# Autodesk Inventor assembly: SolarPanel
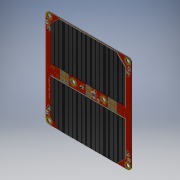
[picture p0: Inventor's stored thumbnail of the model, 180x180]
Saved by Autodesk Inventor 2018 (Build 220112000, 112)
## iProperties
Created: 2018-11-29
Part Number: SolarPanel
Document SubType Name: Assembly
Designer: Bradley
Author: Bradley
## Documents named in this file (32)
- C:\Users\Bradley\Documents\GitHub\CougSat1-Hardware\CougSat1-PowerBoard\CADModel\Native\SolarPanel.iam
- C:\Users\Bradley\Documents\GitHub\CougSat1-Hardware\CougSat1-PowerBoard\CADModel\Native\SolarPanel_PCB.ipt
- C:\Users\Bradley\Documents\GitHub\Resources\SupplierDocuments\04 - Connectors SMT\04-0001\04-0001.iam
- C:\Users\Bradley\Documents\GitHub\Resources\SupplierDocuments\04 - Connectors SMT\04-0007\04-0007.iam
- C:\Users\Bradley\Documents\GitHub\Resources\SupplierDocuments\26 - Resistor Misc\26-0008\26-0008.ipt
- C:\Users\Bradley\Documents\GitHub\Resources\SupplierDocuments\02 - Solar Cell\02-0001\02-0001.ipt
- C:\Users\Bradley\Documents\GitHub\Resources\SupplierDocuments\34 - Inductor 3225 and larger\34-103A\34-103A.ipt
- C:\Users\Bradley\Documents\GitHub\Resources\SupplierDocuments\66 - Sensor\66-0003\66-0003.ipt
- C:\Users\Bradley\Documents\GitHub\Resources\SupplierDocuments\21 - Resistor 1608\21-0000\21-0000.ipt
- C:\Users\Bradley\Documents\GitHub\Resources\SupplierDocuments\21 - Resistor 1608\21-1201\21-1201.ipt
- C:\Users\Bradley\Documents\GitHub\Resources\SupplierDocuments\21 - Resistor 1608\21-1001\21-1001.ipt
- C:\Users\Bradley\Documents\GitHub\Resources\SupplierDocuments\36 - Ferrite\36-152A\36-152A.ipt
- C:\Users\Bradley\Documents\GitHub\Resources\SupplierDocuments\11 - Capacitor Ceramic 1608\11-102A\11-102A.ipt
- C:\Users\Bradley\Documents\GitHub\Resources\SupplierDocuments\21 - Resistor 1608\21-2201\21-2201.ipt
- C:\Users\Bradley\Documents\GitHub\Resources\SupplierDocuments\16 - Capacitor Tantalum SMT\16-475A\16-475A.ipt
- C:\Users\Bradley\Documents\GitHub\Resources\SupplierDocuments\13 - Capacitor Ceramic 3216\13-475A\13-475A.ipt
- C:\Users\Bradley\Documents\GitHub\Resources\SupplierDocuments\23 - Resistor 3216\23-5m00\23-5m00.ipt
- C:\Users\Bradley\Documents\GitHub\Resources\SupplierDocuments\11 - Capacitor Ceramic 1608\11-106A\11-106A.ipt
- C:\Users\Bradley\Documents\GitHub\Resources\SupplierDocuments\13 - Capacitor Ceramic 3216\13-106A\13-106A.ipt
- C:\Users\Bradley\Documents\GitHub\Resources\SupplierDocuments\21 - Resistor 1608\21-1002\21-1002.ipt
- C:\Users\Bradley\Documents\GitHub\Resources\SupplierDocuments\23 - Resistor 3216\23-12m0\23-12m0.ipt
- C:\Users\Bradley\Documents\GitHub\Resources\SupplierDocuments\16 - Capacitor Tantalum SMT\16-476A\16-476A.ipt
- C:\Users\Bradley\Documents\GitHub\Resources\SupplierDocuments\26 - Resistor Misc\26-0005\26-0005.ipt
- C:\Users\Bradley\Documents\GitHub\Resources\SupplierDocuments\11 - Capacitor Ceramic 1608\11-104A\11-104A.ipt
- C:\Users\Bradley\Documents\GitHub\Resources\SupplierDocuments\21 - Resistor 1608\21-3603\21-3603.ipt
- C:\Users\Bradley\Documents\GitHub\Resources\SupplierDocuments\21 - Resistor 1608\21-8203\21-8203.ipt
- C:\Users\Bradley\Documents\GitHub\Resources\SupplierDocuments\27 - Conversion IC\27-0003\27-0003.ipt
- C:\Users\Bradley\Documents\GitHub\Resources\SupplierDocuments\08 - Amplifier (excluding RF)\08-0002\08-0002.ipt
- C:\Users\Bradley\Documents\GitHub\Resources\SupplierDocuments\08 - Amplifier (excluding RF)\08-0004\08-0004.ipt
- C:\Users\Bradley\Documents\GitHub\Resources\SupplierDocuments\53 - Diode Misc\53-0002\53-0002.ipt
- C:\Users\Bradley\Documents\GitHub\Resources\SupplierDocuments\60 - Power IC\60-0001\60-0001.ipt
- C:\Users\Bradley\Documents\GitHub\CougSat1-Hardware\CougSat1-PowerBoard\CADModel\Native\SolarPanel_CellJumper.ipt
## Components (122 placed, 31 different names)
1. 60-0001:2 — Mate:309, Mate:311, Flush:97
2. 60-0001:1 — Mate:308, Flush:96, Mate:310
3. 53-0002:2 — Mate:304, Flush:94, Flush:95
4. 53-0002:1 — Mate:305, Mate:306, Mate:307
5. 08-0004:4 — Mate:299, Flush:92, Flush:93
6. 08-0004:3 — Mate:298, Flush:90, Flush:91
7. 08-0004:2 — Mate:297, Mate:302, Mate:303
8. 08-0004:1 — Mate:296, Mate:300, Mate:301
9. 08-0002:2 — Mate:293, Flush:88, Flush:89
10. 08-0002:1 — Mate:292, Mate:294, Mate:295
11. 27-0003:2 — Mate:289, Mate:291, Flush:87
12. 27-0003:1 — Mate:288, Flush:86, Mate:290
13. 21-8203:2 — Mate:282, Mate:287, Flush:85
14. 21-8203:1 — Mate:281, Mate:285, Mate:286
15. 21-3603:2 — Mate:280, Mate:284, Flush:84
16. 21-3603:1 — Mate:279, Mate:283, Flush:83
17. 11-104A:17 — Mate:255, Mate:278, Flush:82
18. 11-104A:16 — Mate:254, Mate:277, Flush:81
19. 11-104A:15 — Mate:253, Mate:275, Mate:276
20. 11-104A:14 — Mate:252, Mate:273, Mate:274
21. 11-104A:13 — Mate:251, Mate:271, Mate:272
22. 11-104A:12 — Mate:250, Mate:270, Flush:80
23. 11-104A:11 — Mate:249, Mate:268, Mate:269
24. 11-104A:10 — Mate:248, Mate:267, Flush:79
25. 11-104A:9 — Mate:247, Mate:266, Flush:78
26. 11-104A:8 — Mate:246, Mate:264, Mate:265
27. 11-104A:7 — Mate:245, Mate:263, Flush:77
28. 11-104A:6 — Mate:244, Mate:261, Mate:262
29. 11-104A:5 — Mate:243, Mate:260, Flush:76
30. 11-104A:4 — Mate:242, Mate:259, Flush:75
31. 11-104A:3 — Mate:241, Mate:258, Flush:74
32. 11-104A:2 — Mate:240, Mate:257, Flush:73
33. 11-104A:1 — Mate:239, Mate:256, Flush:72
34. 26-0005:2 — Mate:236, Mate:238, Flush:71
35. 26-0005:1 — Mate:235, Mate:237, Flush:70
36. 16-476A:2 — Mate:232, Mate:234, Flush:69
37. 16-476A:1 — Mate:231, Flush:68, Mate:233
38. 23-12m0:2 — Mate:228, Mate:230, Flush:67
39. 23-12m0:1 — Mate:227, Mate:229, Flush:66
40. 26-0008:9 — Mate:212, Mate:225, Mate:226
41. 26-0008:8 — Mate:211, Mate:223, Mate:224
42. 26-0008:7 — Mate:210, Mate:221, Mate:222
43. 26-0008:6 — Mate:209, Mate:219, Mate:220
44. 26-0008:5 — Mate:208, Mate:218, Flush:65
45. 26-0008:4 — Mate:207, Mate:217, Flush:64
46. 26-0008:3 — Mate:206, Mate:215, Mate:216
47. 26-0008:2 — Mate:205, Mate:214, Flush:63
48. 26-0008:1 — Mate:204, Mate:213, Flush:62
49. 21-1002:11 — Mate:176, Mate:203, Flush:61
50. 21-1002:10 — Mate:177, Mate:202, Flush:60
51. 21-1002:9 — Mate:178, Mate:201, Flush:59
52. 21-1002:8 — Mate:179, Mate:199, Mate:200
53. 21-1002:7 — Mate:180, Mate:197, Mate:198
54. 21-1002:6 — Mate:181, Mate:196, Flush:58
55. 21-1002:5 — Mate:182, Mate:194, Mate:195
56. 21-1002:4 — Mate:183, Mate:192, Mate:193
57. 21-1002:3 — Mate:184, Mate:191, Flush:57
58. 21-1002:2 — Mate:185, Mate:189, Mate:190
59. 21-1002:1 — Mate:186, Mate:187, Mate:188
60. 13-106A:4 — Mate:169, Mate:175, Flush:56
61. 13-106A:3 — Mate:168, Mate:174, Flush:55
62. 13-106A:2 — Mate:167, Mate:173, Flush:54
63. 13-106A:1 — Mate:166, Mate:172, Flush:53
64. 11-106A:2 — Mate:165, Mate:171, Flush:52
65. 11-106A:1 — Mate:164, Mate:170, Flush:51
66. 23-5m00:2 — Mate:161, Mate:162, Mate:163
67. 23-5m00:1 — Mate:160, Flush:49, Flush:50
68. 13-475A:4 — Mate:156, Mate:159, Flush:48
69. 13-475A:3 — Mate:155, Flush:46, Flush:47
70. 13-475A:2 — Mate:154, Flush:44, Flush:45
71. 13-475A:1 — Mate:153, Mate:158, Flush:43
72. 16-475A:1 — Mate:152, Flush:42, Mate:157
73. 21-2201:4 — Mate:144, Mate:151, Flush:41
74. 21-2201:3 — Mate:145, Mate:150, Flush:40
75. 21-2201:2 — Mate:143, Mate:149, Flush:39
76. 21-2201:1 — Mate:142, Mate:148, Flush:38
77. 11-102A:2 — Mate:141, Mate:147, Flush:37
78. 11-102A:1 — Mate:140, Mate:146, Flush:36
79. 36-152A:1 — Mate:130, Mate:131, Flush:35
80. 21-1001:4 — Mate:129, Mate:138, Mate:139
81. 21-1001:3 — Mate:128, Mate:136, Mate:137
82. 21-1001:2 — Mate:127, Mate:134, Mate:135
83. 21-1001:1 — Mate:126, Mate:132, Mate:133
84. 21-1201:1 — Mate:123, Mate:124, Flush:34
85. 21-0000:26 — Mate:56, Mate:60, Mate:61
86. 21-0000:25 — Mate:57, Mate:62, Mate:63
87. 21-0000:24 — Mate:58, Mate:64, Mate:65
88. 21-0000:23 — Mate:59, Mate:66, Mate:67
89. 21-0000:22 — Mate:68, Mate:121, Mate:122
90. 21-0000:21 — Mate:69, Mate:120, Flush:33
91. 21-0000:20 — Mate:70, Mate:118, Mate:119
92. 21-0000:19 — Mate:71, Mate:116, Mate:117
93. 21-0000:18 — Mate:72, Mate:115, Flush:32
94. 21-0000:17 — Mate:73, Mate:114, Flush:31
95. 21-0000:16 — Mate:74, Mate:113, Flush:30
96. 21-0000:15 — Mate:75, Mate:112, Flush:29
97. 21-0000:14 — Mate:76, Mate:110, Mate:111
98. 21-0000:13 — Mate:77, Mate:109, Flush:28
99. 21-0000:12 — Mate:78, Mate:107, Mate:108
100. 21-0000:11 — Mate:79, Mate:105, Mate:106
101. 21-0000:10 — Mate:80, Mate:104, Flush:27
102. 21-0000:9 — Mate:81, Mate:102, Mate:103
103. 21-0000:8 — Mate:82, Mate:100, Mate:101
104. 21-0000:7 — Mate:83, Mate:99, Flush:26
105. 21-0000:6 — Mate:84, Mate:98, Flush:25
106. 21-0000:5 — Mate:85, Mate:97, Flush:24
107. 21-0000:4 — Mate:86, Mate:96, Flush:23
108. 21-0000:3 — Mate:87, Mate:94, Mate:95
109. 21-0000:2 — Mate:88, Mate:92, Mate:93
110. 21-0000:1 — Mate:89, Mate:90, Mate:91
111. 02-0001:1 — Mate:1, Mate:3, Mate:4
112. 02-0001:2 — Mate:2, Flush:1, Flush:2
113. 04-0001:1 [sub-assembly] — Mate:49, Flush:17, Flush:18
114. 04-0007:1 [sub-assembly] — Mate:48, Mate:54, Mate:55
115. 34-103A:1 — Mate:50, Mate:52, Flush:21
116. 34-103A:2 — Mate:51, Mate:53, Flush:22
117. 66-0003:1 — Mate:29, Mate:30, Flush:9
118. SolarPanel_CellJumper:1 — Mate:313, Mate:316, Flush:98
119. SolarPanel_CellJumper:2 — Mate:312, Mate:317, Mate:318, Flush:98
120. SolarPanel_CellJumper:3 — Mate:315, Flush:99, Flush:101
121. SolarPanel_CellJumper:4 — Mate:314, Flush:100, Flush:101, Flush:102
122. SolarPanel_PCB:1 — Mate:1, Mate:2, Mate:29, Mate:48, Mate:49, Mate:50, Mate:51, Mate:56, Mate:57, Mate:58, Mate:59, Mate:68, Mate:69, Mate:70, Mate:71, Mate:72, Mate:73, Mate:74, Mate:75, Mate:76, Mate:77, Mate:78, Mate:79, Mate:80, Mate:81, Mate:82, Mate:83, Mate:84, Mate:85, Mate:86, Mate:87, Mate:88, Mate:89, Mate:123, Mate:126, Mate:127, Mate:128, Mate:129, Mate:130, Mate:140, Mate:141, Mate:142, Mate:143, Mate:144, Mate:145, Mate:152, Mate:153, Mate:154, Mate:155, Mate:156, Mate:160, Mate:161, Mate:164, Mate:165, Mate:166, Mate:167, Mate:168, Mate:169, Mate:176, Mate:177, Mate:178, Mate:179, Mate:180, Mate:181, Mate:182, Mate:183, Mate:184, Mate:185, Mate:186, Mate:204, Mate:205, Mate:206, Mate:207, Mate:208, Mate:209, Mate:210, Mate:211, Mate:212, Mate:227, Mate:228, Mate:231, Mate:232, Mate:235, Mate:236, Mate:239, Mate:240, Mate:241, Mate:242, Mate:243, Mate:244, Mate:245, Mate:246, Mate:247, Mate:248, Mate:249, Mate:250, Mate:251, Mate:252, Mate:253, Mate:254, Mate:255, Mate:279, Mate:280, Mate:281, Mate:282, Mate:288, Mate:289, Mate:292, Mate:293, Mate:296, Mate:297, Mate:298, Mate:299, Mate:304, Mate:305, Mate:308, Mate:309, Mate:312, Mate:313, Mate:314, Mate:315
## Relationships (363: Mate 276, Flush 87)
- Mate:1: 02-0001:1 ↔ SolarPanel_PCB:1
- Mate:2: 02-0001:2 ↔ SolarPanel_PCB:1
- Mate:3: 02-0001:1
- Flush:1: 02-0001:2
- Flush:2 (5 mm): 02-0001:2
- Mate:4 (5 mm): 02-0001:1
- Mate:29: 66-0003:1 ↔ SolarPanel_PCB:1
- Mate:30: 66-0003:1
- Flush:9 (-5.5 mm): 66-0003:1
- Mate:48: 04-0007:1 ↔ SolarPanel_PCB:1
- Mate:49: 04-0001:1 ↔ SolarPanel_PCB:1
- Flush:17 (26 mm): 04-0001:1
- Flush:18 (-2.5 mm): 04-0001:1
- Mate:54 (-23.75 mm): 04-0007:1
- Mate:55 (-2.5 mm): 04-0007:1
- Mate:50: 34-103A:1 ↔ SolarPanel_PCB:1
- Mate:51: 34-103A:2 ↔ SolarPanel_PCB:1
- Mate:52 (-9 mm): 34-103A:1
- Flush:21 (9 mm): 34-103A:1
- Mate:53 (9 mm): 34-103A:2
- Flush:22 (-9 mm): 34-103A:2
- Mate:56: 21-0000:26 ↔ SolarPanel_PCB:1
- Mate:57: 21-0000:25 ↔ SolarPanel_PCB:1
- Mate:58: 21-0000:24 ↔ SolarPanel_PCB:1
- Mate:59: 21-0000:23 ↔ SolarPanel_PCB:1
- Mate:60 (-37.75 mm): 21-0000:26
- Mate:61 (37.25 mm): 21-0000:26
- Mate:62 (37.753 mm): 21-0000:25
- Mate:63 (37.25 mm): 21-0000:25
- Mate:64 (-37.75 mm): 21-0000:24
- Mate:65 (-37.25 mm): 21-0000:24
- Mate:66 (37.75 mm): 21-0000:23
- Mate:67 (-37.5 mm): 21-0000:23
- Mate:68: 21-0000:22 ↔ SolarPanel_PCB:1
- Mate:69: 21-0000:21 ↔ SolarPanel_PCB:1
- Mate:70: 21-0000:20 ↔ SolarPanel_PCB:1
- Mate:71: 21-0000:19 ↔ SolarPanel_PCB:1
- Mate:72: 21-0000:18 ↔ SolarPanel_PCB:1
- Mate:73: 21-0000:17 ↔ SolarPanel_PCB:1
- Mate:74: 21-0000:16 ↔ SolarPanel_PCB:1
- Mate:75: 21-0000:15 ↔ SolarPanel_PCB:1
- Mate:76: 21-0000:14 ↔ SolarPanel_PCB:1
- Mate:77: 21-0000:13 ↔ SolarPanel_PCB:1
- Mate:78: 21-0000:12 ↔ SolarPanel_PCB:1
- Mate:79: 21-0000:11 ↔ SolarPanel_PCB:1
- Mate:80: 21-0000:10 ↔ SolarPanel_PCB:1
- Mate:81: 21-0000:9 ↔ SolarPanel_PCB:1
- Mate:82: 21-0000:8 ↔ SolarPanel_PCB:1
- Mate:83: 21-0000:7 ↔ SolarPanel_PCB:1
- Mate:84: 21-0000:6 ↔ SolarPanel_PCB:1
- Mate:85: 21-0000:5 ↔ SolarPanel_PCB:1
- Mate:86: 21-0000:4 ↔ SolarPanel_PCB:1
- Mate:87: 21-0000:3 ↔ SolarPanel_PCB:1
- Mate:88: 21-0000:2 ↔ SolarPanel_PCB:1
- Mate:89: 21-0000:1 ↔ SolarPanel_PCB:1
- Mate:90 (-17 mm): 21-0000:1
- Mate:91 (8.75 mm): 21-0000:1
- Mate:92 (-16 mm): 21-0000:2
- Mate:93 (-17.25 mm): 21-0000:2
- Mate:94 (-16 mm): 21-0000:3
- Mate:95 (-19 mm): 21-0000:3
- Mate:96 (20 mm): 21-0000:4
- Flush:23 (10.5 mm): 21-0000:4
- Mate:97 (20 mm): 21-0000:5
- Flush:24 (8.75 mm): 21-0000:5
- Mate:98 (17 mm): 21-0000:6
- Flush:25 (10.5 mm): 21-0000:6
- Mate:99 (17 mm): 21-0000:7
- Flush:26 (8.75 mm): 21-0000:7
- Mate:100 (-9 mm): 21-0000:8
- Mate:101 (10.75 mm): 21-0000:8
- Mate:102 (-12 mm): 21-0000:9
- Mate:103 (8 mm): 21-0000:9
- Mate:104 (16.75 mm): 21-0000:10
- Flush:27 (5.25 mm): 21-0000:10
- Mate:105 (1.5 mm): 21-0000:11
- Mate:106 (-3 mm): 21-0000:11
- Mate:107 (3 mm): 21-0000:12
- Mate:108 (-4.75 mm): 21-0000:12
- Mate:109 (-16.75 mm): 21-0000:13
- Flush:28 (-5.25 mm): 21-0000:13
- Mate:110 (9 mm): 21-0000:14
- Mate:111 (-10.75 mm): 21-0000:14
- Mate:112 (-15.25 mm): 21-0000:15
- Flush:29 (-9 mm): 21-0000:15
- Mate:113 (-15.25 mm): 21-0000:16
- Flush:30 (-10.75 mm): 21-0000:16
- Mate:114 (-18.25 mm): 21-0000:17
- Flush:31 (-9 mm): 21-0000:17
- Mate:115 (-18.25 mm): 21-0000:18
- Flush:32 (-10.75 mm): 21-0000:18
- Mate:116 (12 mm): 21-0000:19
- Mate:117 (-8 mm): 21-0000:19
- Mate:118 (13.25 mm): 21-0000:20
- Mate:119 (-13.5 mm): 21-0000:20
- Mate:120 (-15 mm): 21-0000:21
- Flush:33 (-18.75 mm): 21-0000:21
- Mate:121 (22.25 mm): 21-0000:22
- Mate:122 (-20.25 mm): 21-0000:22
- Mate:123: 21-1201:1 ↔ SolarPanel_PCB:1
- Mate:124 (-3 mm): 21-1201:1
- Flush:34 (-9 mm): 21-1201:1
- Mate:126: 21-1001:1 ↔ SolarPanel_PCB:1
- Mate:127: 21-1001:2 ↔ SolarPanel_PCB:1
- Mate:128: 21-1001:3 ↔ SolarPanel_PCB:1
- Mate:129: 21-1001:4 ↔ SolarPanel_PCB:1
- Mate:130: 36-152A:1 ↔ SolarPanel_PCB:1
- Mate:131 (-24.75 mm): 36-152A:1
- Flush:35 (17.75 mm): 36-152A:1
- Mate:132 (-14 mm): 21-1001:1
- Mate:133 (-0.25 mm): 21-1001:1
- Mate:134 (-8.75 mm): 21-1001:2
- Mate:135 (4.25 mm): 21-1001:2
- Mate:136 (8.75 mm): 21-1001:3
- Mate:137 (-4.25 mm): 21-1001:3
- Mate:138 (14 mm): 21-1001:4
- Mate:139 (0.25 mm): 21-1001:4
- Mate:140: 11-102A:1 ↔ SolarPanel_PCB:1
- Mate:141: 11-102A:2 ↔ SolarPanel_PCB:1
- Mate:142: 21-2201:1 ↔ SolarPanel_PCB:1
- Mate:143: 21-2201:2 ↔ SolarPanel_PCB:1
- Mate:144: 21-2201:4 ↔ SolarPanel_PCB:1
- Mate:145: 21-2201:3 ↔ SolarPanel_PCB:1
- Mate:146 (-9 mm): 11-102A:1
- Flush:36 (-9 mm): 11-102A:1
- Mate:147 (9 mm): 11-102A:2
- Flush:37 (-9 mm): 11-102A:2
- Mate:148: 21-2201:1
- Mate:149: 21-2201:2
- Mate:150: 21-2201:3
- Mate:151: 21-2201:4
- Flush:38 (28 mm): 21-2201:1
- Flush:39 (26.25 mm): 21-2201:2
- Flush:40 (23.5 mm): 21-2201:3
- Flush:41 (21.75 mm): 21-2201:4
- Mate:152: 16-475A:1 ↔ SolarPanel_PCB:1
- Mate:153: 13-475A:1 ↔ SolarPanel_PCB:1
- Mate:154: 13-475A:2 ↔ SolarPanel_PCB:1
- Mate:155: 13-475A:3 ↔ SolarPanel_PCB:1
- Mate:156: 13-475A:4 ↔ SolarPanel_PCB:1
- Flush:42 (21.5 mm): 16-475A:1
- Mate:157 (-20.75 mm): 16-475A:1
- Mate:158 (8.5 mm): 13-475A:1
- Flush:43 (-14 mm): 13-475A:1
- Flush:44 (17.75 mm): 13-475A:2
- Flush:45 (6.75 mm): 13-475A:2
- Flush:46 (-17.75 mm): 13-475A:3
- Flush:47 (-6.75 mm): 13-475A:3
- Mate:159 (-8.5 mm): 13-475A:4
- Flush:48 (14 mm): 13-475A:4
- Mate:160: 23-5m00:1 ↔ SolarPanel_PCB:1
- Mate:161: 23-5m00:2 ↔ SolarPanel_PCB:1
- Flush:49 (12.5 mm): 23-5m00:1
- Flush:50 (-5.25 mm): 23-5m00:1
- Mate:162 (12.5 mm): 23-5m00:2
- Mate:163 (-5.25 mm): 23-5m00:2
- Mate:164: 11-106A:1 ↔ SolarPanel_PCB:1
- Mate:165: 11-106A:2 ↔ SolarPanel_PCB:1
- Mate:166: 13-106A:1 ↔ SolarPanel_PCB:1
- Mate:167: 13-106A:2 ↔ SolarPanel_PCB:1
- Mate:168: 13-106A:3 ↔ SolarPanel_PCB:1
- Mate:169: 13-106A:4 ↔ SolarPanel_PCB:1
- Mate:170 (-16 mm): 11-106A:1
- Flush:51 (-16.5 mm): 11-106A:1
- Mate:171 (16.25 mm): 11-106A:2
- Flush:52 (15.25 mm): 11-106A:2
- Mate:172 (-13 mm): 13-106A:1
- Flush:53 (-2 mm): 13-106A:1
- Mate:173 (-8.25 mm): 13-106A:2
- Flush:54 (-2 mm): 13-106A:2
- Mate:174 (8.25 mm): 13-106A:3
- Flush:55 (2 mm): 13-106A:3
- Mate:175 (13 mm): 13-106A:4
- Flush:56 (2 mm): 13-106A:4
- Mate:176: 21-1002:11 ↔ SolarPanel_PCB:1
- Mate:177: 21-1002:10 ↔ SolarPanel_PCB:1
- Mate:178: 21-1002:9 ↔ SolarPanel_PCB:1
- Mate:179: 21-1002:8 ↔ SolarPanel_PCB:1
- Mate:180: 21-1002:7 ↔ SolarPanel_PCB:1
- Mate:181: 21-1002:6 ↔ SolarPanel_PCB:1
- Mate:182: 21-1002:5 ↔ SolarPanel_PCB:1
- Mate:183: 21-1002:4 ↔ SolarPanel_PCB:1
- Mate:184: 21-1002:3 ↔ SolarPanel_PCB:1
- Mate:185: 21-1002:2 ↔ SolarPanel_PCB:1
- Mate:186: 21-1002:1 ↔ SolarPanel_PCB:1
- Mate:187 (-36.5 mm): 21-1002:1
- Mate:188 (33 mm): 21-1002:1
- Mate:189 (36.5 mm): 21-1002:2
- Mate:190 (33 mm): 21-1002:2
- Mate:191: 21-1002:3
- Flush:57 (4.75 mm): 21-1002:3
- Mate:192 (-36.5 mm): 21-1002:4
- Mate:193 (-32.75 mm): 21-1002:4
- Mate:194 (36.5 mm): 21-1002:5
- Mate:195 (-33.25 mm): 21-1002:5
- Mate:196 (-18.75 mm): 21-1002:6
- Flush:58 (30.75 mm): 21-1002:6
- Mate:197 (-8 mm): 21-1002:7
- Mate:198 (-0.25 mm): 21-1002:7
- Mate:199 (8 mm): 21-1002:8
- Mate:200 (0.25 mm): 21-1002:8
- Mate:201 (-23.25 mm): 21-1002:9
- Flush:59 (-15 mm): 21-1002:9
- Mate:202 (-23.25 mm): 21-1002:10
- Flush:60 (-16.75 mm): 21-1002:10
- Mate:203: 21-1002:11
- Flush:61 (-29 mm): 21-1002:11
- Mate:204: 26-0008:1 ↔ SolarPanel_PCB:1
- Mate:205: 26-0008:2 ↔ SolarPanel_PCB:1
- Mate:206: 26-0008:3 ↔ SolarPanel_PCB:1
- Mate:207: 26-0008:4 ↔ SolarPanel_PCB:1
- Mate:208: 26-0008:5 ↔ SolarPanel_PCB:1
- Mate:209: 26-0008:6 ↔ SolarPanel_PCB:1
- Mate:210: 26-0008:7 ↔ SolarPanel_PCB:1
- Mate:211: 26-0008:8 ↔ SolarPanel_PCB:1
- Mate:212: 26-0008:9 ↔ SolarPanel_PCB:1
- Mate:213 (-36.5 mm): 26-0008:1
- Flush:62 (-31.25 mm): 26-0008:1
- Mate:214 (36.5 mm): 26-0008:2
- Flush:63 (-31.25 mm): 26-0008:2
- Mate:215: 26-0008:3
- Mate:216 (-6.5 mm): 26-0008:3
- Mate:217 (-36.5 mm): 26-0008:4
- Flush:64 (31 mm): 26-0008:4
- Mate:218 (36.5 mm): 26-0008:5
- Flush:65 (31.5 mm): 26-0008:5
- Mate:219: 26-0008:6
- Mate:220 (-30.75 mm): 26-0008:6
- Mate:221 (-7.5 mm): 26-0008:7
- Mate:222 (-14 mm): 26-0008:7
- Mate:223 (8 mm): 26-0008:8
- Mate:224 (14.25 mm): 26-0008:8
- Mate:225: 26-0008:9
- Mate:226 (30.75 mm): 26-0008:9
- Mate:227: 23-12m0:1 ↔ SolarPanel_PCB:1
- Mate:228: 23-12m0:2 ↔ SolarPanel_PCB:1
- Mate:229 (-17.75 mm): 23-12m0:1
- Flush:66 (9.5 mm): 23-12m0:1
- Mate:230 (18 mm): 23-12m0:2
- Flush:67 (-9.5 mm): 23-12m0:2
- Mate:231: 16-476A:1 ↔ SolarPanel_PCB:1
- Mate:232: 16-476A:2 ↔ SolarPanel_PCB:1
- Flush:68 (8.25 mm): 16-476A:1
- Mate:233 (-22.25 mm): 16-476A:1
- Mate:234 (8.25 mm): 16-476A:2
- Flush:69 (-22.25 mm): 16-476A:2
- Mate:235: 26-0005:1 ↔ SolarPanel_PCB:1
- Mate:236: 26-0005:2 ↔ SolarPanel_PCB:1
- Mate:237 (-18 mm): 26-0005:1
- Flush:70 (-19.25 mm): 26-0005:1
- Mate:238 (-20.75 mm): 26-0005:2
- Flush:71 (-19.25 mm): 26-0005:2
- Mate:239: 11-104A:1 ↔ SolarPanel_PCB:1
- Mate:240: 11-104A:2 ↔ SolarPanel_PCB:1
- Mate:241: 11-104A:3 ↔ SolarPanel_PCB:1
- Mate:242: 11-104A:4 ↔ SolarPanel_PCB:1
- Mate:243: 11-104A:5 ↔ SolarPanel_PCB:1
- Mate:244: 11-104A:6 ↔ SolarPanel_PCB:1
- Mate:245: 11-104A:7 ↔ SolarPanel_PCB:1
- Mate:246: 11-104A:8 ↔ SolarPanel_PCB:1
- Mate:247: 11-104A:9 ↔ SolarPanel_PCB:1
- Mate:248: 11-104A:10 ↔ SolarPanel_PCB:1
- Mate:249: 11-104A:11 ↔ SolarPanel_PCB:1
- Mate:250: 11-104A:12 ↔ SolarPanel_PCB:1
- Mate:251: 11-104A:13 ↔ SolarPanel_PCB:1
- Mate:252: 11-104A:14 ↔ SolarPanel_PCB:1
- Mate:253: 11-104A:15 ↔ SolarPanel_PCB:1
- Mate:254: 11-104A:16 ↔ SolarPanel_PCB:1
- Mate:255: 11-104A:17 ↔ SolarPanel_PCB:1
- Mate:256 (-37.75 mm): 11-104A:1
- Flush:72 (-35.5 mm): 11-104A:1
- Mate:257 (37.75 mm): 11-104A:2
- Flush:73 (-35.5 mm): 11-104A:2
- Mate:258 (-37.75 mm): 11-104A:3
- Flush:74 (35.25 mm): 11-104A:3
- Mate:259 (37.75 mm): 11-104A:4
- Flush:75 (35.75 mm): 11-104A:4
- Mate:260 (-21.75 mm): 11-104A:5
- Flush:76 (17.75 mm): 11-104A:5
- Mate:261 (14 mm): 11-104A:6
- Mate:262 (-13.75 mm): 11-104A:6
- Mate:263 (-17 mm): 11-104A:7
- Flush:77 (-10.5 mm): 11-104A:7
- Mate:264 (23 mm): 11-104A:8
- Mate:265 (-10.5 mm): 11-104A:8
- Mate:266 (-13 mm): 11-104A:9
- Flush:78 (-16.5 mm): 11-104A:9
- Mate:267 (-11 mm): 11-104A:10
- Flush:79 (0.25 mm): 11-104A:10
- Mate:268 (13.75 mm): 11-104A:11
- Mate:269 (-5.25 mm): 11-104A:11
- Mate:270 (11 mm): 11-104A:12
- Flush:80 (-0.25 mm): 11-104A:12
- Mate:271 (-16.75 mm): 11-104A:13
- Mate:272 (7 mm): 11-104A:13
- Mate:273 (-21.25 mm): 11-104A:14
- Mate:274 (10.75 mm): 11-104A:14
- Mate:275 (-11 mm): 11-104A:15
- Mate:276 (14 mm): 11-104A:15
- Mate:277 (13.25 mm): 11-104A:16
- Flush:81 (15.25 mm): 11-104A:16
- Mate:278 (18 mm): 11-104A:17
- Flush:82 (8.5 mm): 11-104A:17
- Mate:279: 21-3603:1 ↔ SolarPanel_PCB:1
- Mate:280: 21-3603:2 ↔ SolarPanel_PCB:1
- Mate:281: 21-8203:1 ↔ SolarPanel_PCB:1
- Mate:282: 21-8203:2 ↔ SolarPanel_PCB:1
- Mate:283 (9.5 mm): 21-3603:1
- Flush:83 (6.5 mm): 21-3603:1
- Mate:284 (-9.5 mm): 21-3603:2
- Flush:84 (-6.5 mm): 21-3603:2
- Mate:285 (-12 mm): 21-8203:1
- Mate:286 (9.75 mm): 21-8203:1
- Mate:287 (-10.5 mm): 21-8203:2
- Flush:85 (-11.5 mm): 21-8203:2
- Mate:288: 27-0003:1 ↔ SolarPanel_PCB:1
- Mate:289: 27-0003:2 ↔ SolarPanel_PCB:1
- Flush:86 (14.25 mm): 27-0003:1
- Mate:290 (20.25 mm): 27-0003:1
- Mate:291 (14.5 mm): 27-0003:2
- Flush:87 (19 mm): 27-0003:2
- Mate:292: 08-0002:1 ↔ SolarPanel_PCB:1
- Mate:293: 08-0002:2 ↔ SolarPanel_PCB:1
- Mate:294 (13.5 mm): 08-0002:1
- Mate:295 (-17 mm): 08-0002:1
- Flush:88 (11.5 mm): 08-0002:2
- Flush:89 (-17.25 mm): 08-0002:2
- Mate:296: 08-0004:1 ↔ SolarPanel_PCB:1
- Mate:297: 08-0004:2 ↔ SolarPanel_PCB:1
- Mate:298: 08-0004:3 ↔ SolarPanel_PCB:1
- Mate:299: 08-0004:4 ↔ SolarPanel_PCB:1
- Mate:300 (5 mm): 08-0004:1
- Mate:301 (-16.5 mm): 08-0004:1
- Mate:302 (-17.75 mm): 08-0004:2
- Mate:303 (-12.5 mm): 08-0004:2
- Flush:90 (-17.75 mm): 08-0004:3
- Flush:91 (-12.5 mm): 08-0004:3
- Flush:92 (5 mm): 08-0004:4
- Flush:93 (-16.5 mm): 08-0004:4
- Mate:304: 53-0002:2 ↔ SolarPanel_PCB:1
- Mate:305: 53-0002:1 ↔ SolarPanel_PCB:1
- Mate:306 (-8 mm): 53-0002:1
- Mate:307 (6.5 mm): 53-0002:1
- Flush:94 (-8 mm): 53-0002:2
- Flush:95 (6.5 mm): 53-0002:2
- Mate:308: 60-0001:1 ↔ SolarPanel_PCB:1
- Mate:309: 60-0001:2 ↔ SolarPanel_PCB:1
- Flush:96 (9.75 mm): 60-0001:1
- Mate:310 (-3.25 mm): 60-0001:1
- Mate:311 (9.75 mm): 60-0001:2
- Flush:97 (-3.25 mm): 60-0001:2
- Mate:312: SolarPanel_CellJumper:2 ↔ SolarPanel_PCB:1
- Mate:313: SolarPanel_CellJumper:1 ↔ SolarPanel_PCB:1
- Mate:314: SolarPanel_CellJumper:4 ↔ SolarPanel_PCB:1
- Mate:315: SolarPanel_CellJumper:3 ↔ SolarPanel_PCB:1
- Mate:316 (27 mm): SolarPanel_CellJumper:1
- Mate:317 (-27 mm): SolarPanel_CellJumper:2
- Mate:318 (19.5 mm): SolarPanel_CellJumper:2
- Flush:98: SolarPanel_CellJumper:1 ↔ SolarPanel_CellJumper:2
- Flush:99 (27 mm): SolarPanel_CellJumper:3
- Flush:100 (-27 mm): SolarPanel_CellJumper:4
- Flush:101: SolarPanel_CellJumper:3 ↔ SolarPanel_CellJumper:4
- Flush:102 (19.5 mm): SolarPanel_CellJumper:4
